# Autodesk Inventor assembly: Goals
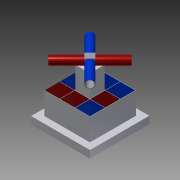
[picture p0: Inventor's stored thumbnail of the model, 180x180]
Saved by Autodesk Inventor 2014 (Build 180170000, 170)
## iProperties
Created: 2014-12-02
Part Number: Goals
Document SubType Name: Assembly
Designer: vandenrobots
Author: vandenrobots
## Documents named in this file (3)
- \\DRAFTSERVER\robotics\Green Games\Goals.iam
- \\DRAFTSERVER\robotics\Green Games\Horizontal Goals.ipt
- \\DRAFTSERVER\robotics\Green Games\Vertical Goals.ipt
## Components (2 placed, 2 different names)
1. Horizontal Goals:1 — Tangent:1, Tangent:2, Angle:1, Mate:1, Mate:2
2. Vertical Goals:1 — Tangent:1, Tangent:2, Angle:1, Mate:1, Mate:2
## Relationships (5: Tangent 2, Mate 2, Angle 1)
- Tangent:1: Horizontal Goals:1 ↔ Vertical Goals:1
- Tangent:2: Horizontal Goals:1 ↔ Vertical Goals:1
- Angle:1 (45 deg): Horizontal Goals:1 ↔ Vertical Goals:1
- Mate:1 (-304.8 mm): Horizontal Goals:1 ↔ Vertical Goals:1
- Mate:2 (-304.8 mm): Horizontal Goals:1 ↔ Vertical Goals:1
